# Autodesk Inventor assembly: PistonLift-ver1-1111-2020
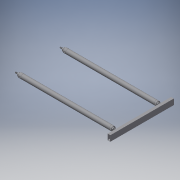
[picture p0: Inventor's stored thumbnail of the model, 180x180]
Saved by Autodesk Inventor 2018 (Build 220112000, 112)
## iProperties
Created: 2020-01-25
Part Number: PistonLift-ver1-1111-2020
Document SubType Name: Assembly
Designer: JMHal
Author: JMHal
## Documents named in this file (3)
- E:\GrabCAD\Power Hawks CAD\2020 Infinite Recharge\Lift\Assemblies\PistonLift-ver1-1111-2020.iam
- E:\GrabCAD\Power Hawks CAD\2020 Infinite Recharge\Lift\Parts\1.5_Bore_30in_Stroke_ROUND BODY AIR CYLINDER.iam
- E:\GrabCAD\Power Hawks CAD\2020 Infinite Recharge\Lift\Parts\PistonMount.ipt
## Components (3 placed, 2 different names)
1. 1.5_Bore_30in_Stroke_ROUND BODY AIR CYLINDER:1 [sub-assembly] — Mate:1, Flush:2
2. 1.5_Bore_30in_Stroke_ROUND BODY AIR CYLINDER:2 [sub-assembly] — Mate:2, Flush:1
3. PistonMount:1 — Mate:1, Mate:2, Mate:3, Mate:4, Flush:1, Flush:2
## Relationships (6: Mate 4, Flush 2)
- Mate:1 (25.4 mm): 1.5_Bore_30in_Stroke_ROUND BODY AIR CYLINDER:1 ↔ PistonMount:1
- Mate:2 (25.4 mm): 1.5_Bore_30in_Stroke_ROUND BODY AIR CYLINDER:2 ↔ PistonMount:1
- Mate:3: PistonMount:1
- Mate:4: PistonMount:1
- Flush:1 (-76.2 mm): 1.5_Bore_30in_Stroke_ROUND BODY AIR CYLINDER:2 ↔ PistonMount:1
- Flush:2 (-76.2 mm): 1.5_Bore_30in_Stroke_ROUND BODY AIR CYLINDER:1 ↔ PistonMount:1
